# Autodesk Inventor assembly: Pr1
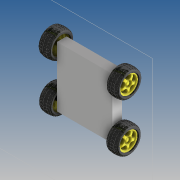
[picture p0: Inventor's stored thumbnail of the model, 180x180]
Saved by Autodesk Inventor 2020 (Build 240168000, 168)
## iProperties
Created: 2019-12-03
Part Number: Pr1
Document SubType Name: Assembly
Designer: Berkant
Author: Berkant
## Documents named in this file (4)
- C:\Users\berka\Desktop\School\Project 2\Prototype 1\Pr1.iam
- C:\Users\berka\Desktop\School\Project 2\prototype 1.ipt
- C:\Users\berka\Desktop\Arduino Gear Motor.ipt
- C:\Users\berka\Desktop\wheel (scaled).ipt
## Components (9 placed, 3 different names)
1. prototype 1:1 — Rigid:1, Rigid:2, Rigid:3, Rigid:4
2. Arduino Gear Motor:1 — Rigid:3, Rotational:3
3. Arduino Gear Motor:5 — Rigid:2, Rotational:2
4. Arduino Gear Motor:6 — Rigid:4, Rigid:5
5. Arduino Gear Motor:7 — Rigid:1, Rotational:1
6. wheel (scaled):2 — Rotational:1
7. wheel (scaled):3 — Rotational:2
8. wheel (scaled):4 — Rotational:3
9. wheel (scaled):5 — Rigid:5
## Relationships (8: WeldJoint 5, RevoluteJoint 3)
- Rigid:1 [WeldJoint]: prototype 1:1 ↔ Arduino Gear Motor:7
- Rigid:2 [WeldJoint]: prototype 1:1 ↔ Arduino Gear Motor:5
- Rigid:3 [WeldJoint]: prototype 1:1 ↔ Arduino Gear Motor:1
- Rigid:4 [WeldJoint]: prototype 1:1 ↔ Arduino Gear Motor:6
- Rotational:1 [RevoluteJoint] (4 mm): Arduino Gear Motor:7 ↔ wheel (scaled):2
- Rotational:2 [RevoluteJoint] (8 mm): Arduino Gear Motor:5 ↔ wheel (scaled):3
- Rigid:5 [WeldJoint] (4 mm): Arduino Gear Motor:6 ↔ wheel (scaled):5
- Rotational:3 [RevoluteJoint] (8 mm): Arduino Gear Motor:1 ↔ wheel (scaled):4
